# Autodesk Inventor assembly: bin_modified_assembly
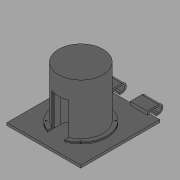
[picture p0: Inventor's stored thumbnail of the model, 180x180]
Saved by Autodesk Inventor 2019 (Build 230136000, 136)
## iProperties
Part Number: bin_modified_assembly
Document SubType Name: Assembly
Designer: Javi
Author: Javi
## Documents named in this file (9)
- D:\MisterBin\bin_modified_assembly.iam
- D:\MisterBin\bin_lid_addon.ipt
- D:\MisterBin\bin_modified.ipt
- D:\MisterBin\inner_mechanism.ipt
- D:\MisterBin\mechanism_cover.ipt
- D:\MisterBin\external_cover.ipt
- D:\MisterBin\rfid_cover.ipt
- D:\MisterBin\Parallax-Servo_DUMMY.ipt
- D:\MisterBin\Parallax-Servo-Horn.ipt
## Components (8 placed, 8 different names)
1. bin_modified:1 — Rotational:1, Mate:1
2. bin_lid_addon:1 — Rotational:1, Rotational:2, Mate:1, Insert:1, Insert:2, Slider:1
3. inner_mechanism:1 — Rotational:2
4. mechanism_cover:1 — Insert:1, Insert:2, Insert:3, Insert:4, Insert:5, Insert:6
5. external_cover:1 — Insert:3, Insert:4
6. rfid_cover:1 — Slider:1
7. Parallax-Servo_DUMMY:1 — Rotational:3, Insert:5, Insert:6
8. Parallax-Servo-Horn:1 — Rotational:3
## Relationships (11: Insert 6, RevoluteJoint 3, Mate 1, TranslationJoint 1)
- Rotational:1 [RevoluteJoint] (6 mm): bin_modified:1 ↔ bin_lid_addon:1
- Rotational:2 [RevoluteJoint]: bin_lid_addon:1 ↔ inner_mechanism:1
- Mate:1: bin_modified:1 ↔ bin_lid_addon:1
- Insert:1: bin_lid_addon:1 ↔ mechanism_cover:1
- Insert:2: bin_lid_addon:1 ↔ mechanism_cover:1
- Insert:3: mechanism_cover:1 ↔ external_cover:1
- Insert:4: mechanism_cover:1 ↔ external_cover:1
- Rotational:3 [RevoluteJoint]: Parallax-Servo_DUMMY:1 ↔ Parallax-Servo-Horn:1
- Slider:1 [TranslationJoint]: bin_lid_addon:1 ↔ rfid_cover:1
- Insert:5 (2 mm): mechanism_cover:1 ↔ Parallax-Servo_DUMMY:1
- Insert:6 (2 mm): mechanism_cover:1 ↔ Parallax-Servo_DUMMY:1
